# Autodesk Inventor assembly: scissor-assembly
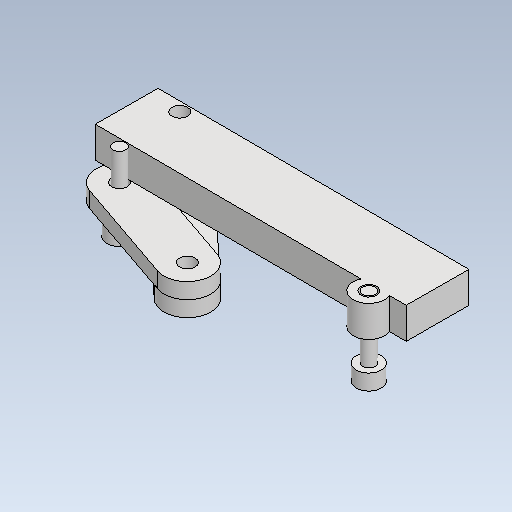
[picture p0: Inventor's stored thumbnail of the model, 512x512]
Saved by Autodesk Inventor 2025 (Build 290162000, 162)
## iProperties
Created: 2025-08-20
Part Number: scissor-assembly
Document SubType Name: Assembly
Designer: HP
Author: HP
## Documents named in this file (5)
- C:\Users\HP\Documents\GitHub\robotics-dojo-2025\CAD\scissor-assembly.iam
- C:\Users\HP\Documents\GitHub\robotics-dojo-2025\CAD\scissor-link.ipt
- C:\Users\HP\Documents\GitHub\robotics-dojo-2025\CAD\temp-pin.ipt
- C:\Users\HP\Documents\GitHub\robotics-dojo-2025\CAD\temp-bed.ipt
- C:\Users\HP\Documents\GitHub\robotics-dojo-2025\CAD\scissor-link-upper.ipt
## Components (5 placed, 4 different names)
1. scissor-link:2 — Mate:3, Flush:1, Mate:6, Mate:7
2. temp-pin:1 — Mate:3, Flush:1, Flush:2, Flush:3, Flush:4
3. temp-bed:1 — Mate:4, Flush:5, Mate:5
4. temp-pin:2 — Flush:2, Flush:3, Flush:4, Mate:4, Flush:5
5. scissor-link-upper:1 — Mate:5, Mate:6, Mate:7
## Relationships (10: Mate 5, Flush 5)
- Mate:3: scissor-link:2 ↔ temp-pin:1
- Flush:1 (10 mm): scissor-link:2 ↔ temp-pin:1
- Flush:2: temp-pin:1 ↔ temp-pin:2
- Flush:3: temp-pin:1 ↔ temp-pin:2
- Flush:4 (80 mm): temp-pin:1 ↔ temp-pin:2
- Mate:4: temp-bed:1 ↔ temp-pin:2
- Flush:5: temp-bed:1 ↔ temp-pin:2
- Mate:5: temp-bed:1 ↔ scissor-link-upper:1
- Mate:6: scissor-link:2 ↔ scissor-link-upper:1
- Mate:7: scissor-link:2 ↔ scissor-link-upper:1
